# Autodesk Inventor assembly: Drawer_WIZ
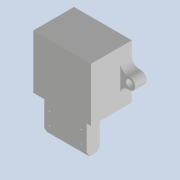
[picture p0: Inventor's stored thumbnail of the model, 180x180]
Saved by Autodesk Inventor 2021 (Build 250183000, 183)
## iProperties
Created: 2025-11-29
Part Number: Drawer_WIZ
Document SubType Name: Assembly
Designer: huber
Sending System: Autodesk Inventor 2026
Preprocessor: ST-DEVELOPER v20.1
Title: Drawer.stp
Author: Miki
## Documents named in this file (4)
- C:\Users\huber\OneDrive\Pulpit\hackaton BHL\BHL 2025\Drawer_WIZ.iam
- C:\Users\huber\OneDrive\Pulpit\hackaton BHL\BHL 2025\Ultrasonic sensor.ipt
- C:\Users\huber\OneDrive\Pulpit\hackaton BHL\BHL 2025\Szuflada.ipt
- C:\Users\huber\OneDrive\Pulpit\hackaton BHL\BHL 2025\sensorBox_WIZ.ipt
## Components (3 placed, 3 different names)
1. Ultrasonic sensor:1 — Mate:3, Mate:4, Mate:5
2. Szuflada:1 — Mate:3, Mate:4, Mate:5, Mate:6, Mate:7, Mate:8
3. sensorBox_WIZ:1 — Mate:6, Mate:7, Mate:8
## Relationships (6: Mate 6)
- Mate:3: Ultrasonic sensor:1 ↔ Szuflada:1
- Mate:4: Ultrasonic sensor:1 ↔ Szuflada:1
- Mate:5: Ultrasonic sensor:1 ↔ Szuflada:1
- Mate:6 (0.5 mm): Szuflada:1 ↔ sensorBox_WIZ:1
- Mate:7: Szuflada:1 ↔ sensorBox_WIZ:1
- Mate:8: Szuflada:1 ↔ sensorBox_WIZ:1
